# Autodesk Inventor assembly: Front Assamblied
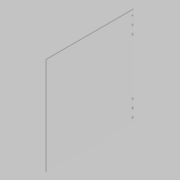
[picture p0: Inventor's stored thumbnail of the model, 180x180]
Saved by Autodesk Inventor 2020 (Build 240168000, 168)
## iProperties
Created: 2020-08-05
Part Number: Front Assamblied
Document SubType Name: Assembly
Designer: Abbas
Author: Abbas
## Documents named in this file (3)
- C:\Users\LENOVO\Desktop\Graduation Project\Fish Farming Unit\Electric Box\Front Assamblied.iam
- C:\Users\LENOVO\Desktop\Graduation Project\Fish Farming Unit\Electric Box\Front.ipt
- C:\Users\LENOVO\Desktop\Graduation Project\Fish Farming Unit\Electric Box\Peice 2.ipt
## Components (3 placed, 2 different names)
1. Front:2 — Mate:1, Insert:1, Mate:2, Insert:2
2. Peice 2:1 — Mate:1, Insert:1
3. Peice 2:2 — Mate:2, Insert:2
## Relationships (4: Mate 2, Insert 2)
- Mate:1: Front:2 ↔ Peice 2:1
- Insert:1: Front:2 ↔ Peice 2:1
- Mate:2: Front:2 ↔ Peice 2:2
- Insert:2: Front:2 ↔ Peice 2:2
